# Autodesk Inventor assembly: module_command
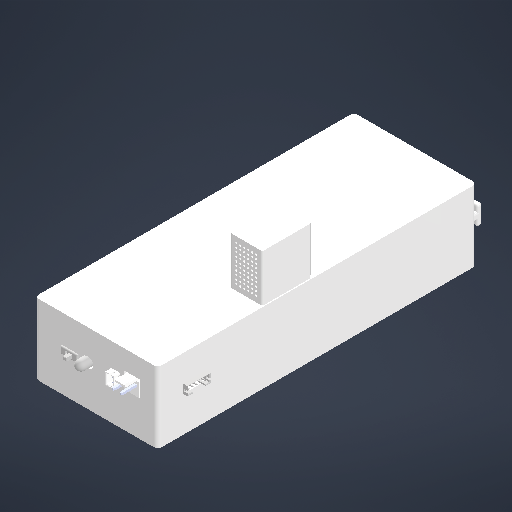
[picture p0: Inventor's stored thumbnail of the model, 512x512]
Saved by Autodesk Inventor 2025.4 (Build 294407000, 407)
## iProperties
Created: 2025-11-12
Part Number: module_command
Document SubType Name: Assembly
Designer: sam
Author: sam
## Documents named in this file (13)
- G:\projects\primary\regulated-irrigation-system\model\asm\module-command\module_command.iam
- G:\projects\primary\regulated-irrigation-system\model\asm\module-command\module_command.ipt
- G:\projects\primary\regulated-irrigation-system\model\asm\module-command\module-lid_command.ipt
- G:\projects\primary\regulated-irrigation-system\model\asm\electronic-components\pcb_command-module.iam
- G:\projects\primary\regulated-irrigation-system\model\asm\electronic-components\battery-5050100_4000.ipt
- G:\projects\primary\regulated-irrigation-system\model\asm\module-command\clip_pcb-command.ipt
- G:\projects\primary\regulated-irrigation-system\model\asm\electronic-components\boost-converter.ipt
- G:\projects\primary\regulated-irrigation-system\model\asm\electronic-components\charge-controller.ipt
- G:\projects\primary\regulated-irrigation-system\model\asm\electronic-components\jst-vh-2p_straight.iam
- G:\projects\primary\regulated-irrigation-system\model\asm\module-command\clip_zs042-command.ipt
- G:\projects\primary\regulated-irrigation-system\model\asm\electronic-components\zs042\ZS042.ipt
- G:\projects\primary\regulated-irrigation-system\model\asm\module-command\encloser-dht22_command.ipt
- G:\projects\primary\regulated-irrigation-system\model\asm\electronic-components\jst-ph-2p\jst-ph-2p.iam
## Components (13 placed, 12 different names)
1. module_command:1 — Mate:3, Mate:4, Mate:5, Mate:6, Mate:7, Mate:12, Mate:14, Mate:15, Mate:16, Mate:19, Mate:20, Mate:21, Mate:22, Flush:1, Flush:2, Flush:3, Mate:23, Mate:24, Mate:25, Mate:32, Mate:33, Mate:34, Flush:4, Mate:35, Mate:36, Mate:37, Mate:38
2. module-lid_command:1 — Flush:2, Flush:3, Mate:29, Mate:30, Mate:31, Mate:32
3. pcb_command-module:1 [sub-assembly] — Mate:9, Mate:10, Mate:11
4. battery-5050100_4000:1 — Mate:3, Mate:4, Mate:5
5. clip_pcb-command:1 — Mate:6, Mate:7, Mate:9, Mate:10, Mate:11, Mate:35
6. boost-converter:1 — Mate:15, Mate:16, Mate:37
7. boost-converter:2 — Mate:12, Mate:14, Mate:38
8. charge-controller:1 — Mate:19, Mate:20, Mate:36
9. jst-vh-2p_straight:1 [sub-assembly] — Mate:21, Mate:22, Flush:1
10. clip_zs042-command:1 — Mate:23, Mate:24, Mate:25, Mate:26, Mate:27, Mate:28
11. ZS042:1 — Mate:26, Mate:27, Mate:28
12. encloser-dht22_command:1 — Mate:29, Mate:30, Mate:31
13. jst-ph-2p:1 [sub-assembly] — Mate:33, Mate:34, Flush:4
## Relationships (36: Mate 32, Flush 4)
- Mate:3: module_command:1 ↔ battery-5050100_4000:1
- Mate:4 (0.2 mm): module_command:1 ↔ battery-5050100_4000:1
- Mate:5 (0.2 mm): module_command:1 ↔ battery-5050100_4000:1
- Mate:6: module_command:1 ↔ clip_pcb-command:1
- Mate:7 (0.2 mm): module_command:1 ↔ clip_pcb-command:1
- Mate:9 (0.2 mm): pcb_command-module:1 ↔ clip_pcb-command:1
- Mate:10: pcb_command-module:1 ↔ clip_pcb-command:1
- Mate:11 (0.2 mm): pcb_command-module:1 ↔ clip_pcb-command:1
- Mate:12 (0.2 mm): module_command:1 ↔ boost-converter:2
- Mate:14: module_command:1 ↔ boost-converter:2
- Mate:15: module_command:1 ↔ boost-converter:1
- Mate:16 (0.2 mm): module_command:1 ↔ boost-converter:1
- Mate:19 (0.2 mm): module_command:1 ↔ charge-controller:1
- Mate:20: module_command:1 ↔ charge-controller:1
- Mate:21 (0.1 mm): module_command:1 ↔ jst-vh-2p_straight:1
- Mate:22 (0.1 mm): module_command:1 ↔ jst-vh-2p_straight:1
- Flush:1: module_command:1 ↔ jst-vh-2p_straight:1
- Flush:2: module_command:1 ↔ module-lid_command:1
- Flush:3: module_command:1 ↔ module-lid_command:1
- Mate:23: module_command:1 ↔ clip_zs042-command:1
- Mate:24 (0.2 mm): module_command:1 ↔ clip_zs042-command:1
- Mate:25 (0.2 mm): module_command:1 ↔ clip_zs042-command:1
- Mate:26 (0.1 mm): clip_zs042-command:1 ↔ ZS042:1
- Mate:27 (0.2 mm): clip_zs042-command:1 ↔ ZS042:1
- Mate:28: clip_zs042-command:1 ↔ ZS042:1
- Mate:29 (0.1 mm): module-lid_command:1 ↔ encloser-dht22_command:1
- Mate:30 (0.1 mm): module-lid_command:1 ↔ encloser-dht22_command:1
- Mate:31: module-lid_command:1 ↔ encloser-dht22_command:1
- Mate:32: module_command:1 ↔ module-lid_command:1
- Mate:33 (0.1 mm): module_command:1 ↔ jst-ph-2p:1
- Mate:34 (0.1 mm): module_command:1 ↔ jst-ph-2p:1
- Flush:4: module_command:1 ↔ jst-ph-2p:1
- Mate:35 (0.2 mm): module_command:1 ↔ clip_pcb-command:1
- Mate:36 (0.2 mm): module_command:1 ↔ charge-controller:1
- Mate:37 (0.2 mm): module_command:1 ↔ boost-converter:1
- Mate:38 (0.2 mm): module_command:1 ↔ boost-converter:2
